# Autodesk Inventor assembly: sestava tělo estonsko pouze s plechem
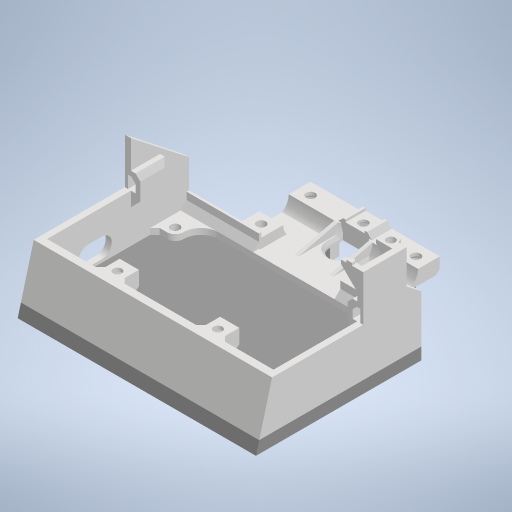
[picture p0: Inventor's stored thumbnail of the model, 512x512]
Saved by Autodesk Inventor 2024 (Build 280153000, 153)
## iProperties
Created: 2023-11-13
Part Number: sestava tělo estonsko pouze s plechem
Document SubType Name: Assembly
Designer: Simak
Author: Simak
## Documents named in this file (3)
- C:\Users\Simak\OneDrive\Dokumenty\GitHub\RoboCop\- 3D -\wip\Tělo s plechem\sestava tělo estonsko pouze s plechem.iam
- C:\Users\Simak\OneDrive\Dokumenty\GitHub\RoboCop\- 3D -\wip\Tělo s plechem\tělo estonsko s plechem otočené motory.ipt
- C:\Users\Simak\OneDrive\Dokumenty\GitHub\RoboCop\- 3D -\mech._parts\plech.ipt
## Components (2 placed, 2 different names)
1. tělo estonsko s plechem otočené motory:1 — Proti sobě:1, Stejný směr:1, Stejný směr:2
2. plech:1 — Proti sobě:1, Stejný směr:1, Stejný směr:2
## Relationships (3: Flush 2, Mate 1)
- Proti sobě:1 [Mate]: tělo estonsko s plechem otočené motory:1 ↔ plech:1
- Stejný směr:1 [Flush]: tělo estonsko s plechem otočené motory:1 ↔ plech:1
- Stejný směr:2 [Flush]: tělo estonsko s plechem otočené motory:1 ↔ plech:1
